# Autodesk Inventor assembly: gear_shaft
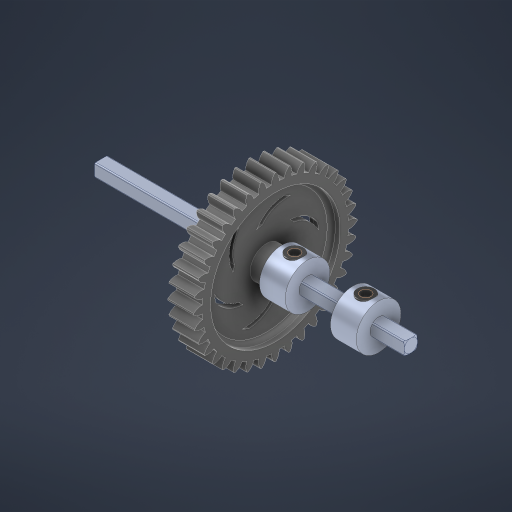
[picture p0: Inventor's stored thumbnail of the model, 512x512]
Saved by Autodesk Inventor 2024 (Build 280153000, 153)
## iProperties
Created: 2024-01-15
Part Number: gear_shaft
Document SubType Name: Assembly
Designer: avere
Author: avere
## Documents named in this file (7)
- C:\Users\avere\Documents\rbp_cad\zoomba_v0.3\chassis\drivebay\gear_shaft.iam
- C:\Users\avere\Documents\rbp_cad\VEX-CAD-Inventor-1.41\Motion\Spacers\Washer Steel\SWasher .375 OD x .062500.ipt
- C:\Users\avere\Documents\rbp_cad\VEX-CAD-Inventor-1.41\Motion\Spacers\Washer Steel.ipt
- C:\Users\avere\Documents\rbp_cad\VEX-CAD-Inventor-1.41\Motion\Gears\LS 36T Gear.ipt
- C:\Users\avere\Documents\rbp_cad\VEX-CAD-Inventor-1.41\Motion\Shaft LS\Shaft Collar ipts\Shaft Collar Set Screw.ipt
- C:\Users\avere\Documents\rbp_cad\VEX-CAD-Inventor-1.41\Motion\Shaft LS\Shaft LS\Shaft LS 3.0.ipt
- C:\Users\avere\Documents\rbp_cad\VEX-CAD-Inventor-1.41\Motion\Shaft LS\Shaft LS.ipt
## Components (5 placed, 4 different names)
1. SWasher .375 OD x .062500:1 — Insert:1
2. LS 36T Gear:1 — Insert:1, Insert:2
3. Shaft Collar Set Screw:1 — Insert:2, Insert:3
4. Shaft Collar Set Screw:2 — Insert:3, Insert:4
5. Shaft LS 3.0:1 — Insert:4
## Relationships (4: Insert 4)
- Insert:1: SWasher .375 OD x .062500:1 ↔ LS 36T Gear:1
- Insert:2: LS 36T Gear:1 ↔ Shaft Collar Set Screw:1
- Insert:3 (11.1125 mm): Shaft Collar Set Screw:1 ↔ Shaft Collar Set Screw:2
- Insert:4 (-7.9375 mm): Shaft Collar Set Screw:2 ↔ Shaft LS 3.0:1
